# Autodesk Inventor assembly: ImpresionGrua
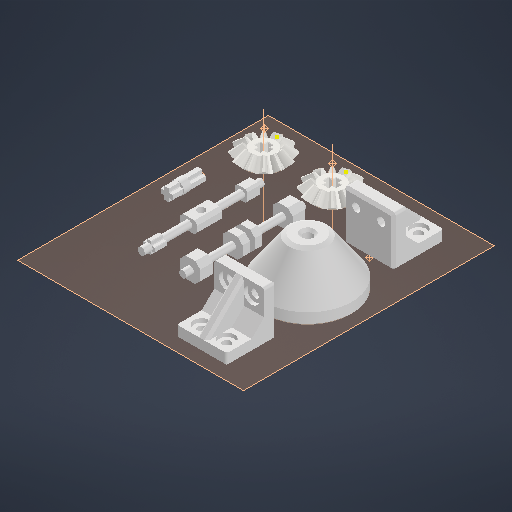
[picture p0: Inventor's stored thumbnail of the model, 512x512]
Saved by Autodesk Inventor 2026.3 (Build 303398000, 398)
## iProperties
Created: 2026-05-15
Part Number: ImpresionGrua
Document SubType Name: Assembly
Designer: Caro
Author: Caro
## Documents named in this file (7)
- C:\Users\Caro\JoseCarlos\TEC\TFG\Inventor\PiezasSTD\EnsamblesDeImpresion\ImpresionGrua.iam
- C:\Users\Caro\JoseCarlos\TEC\TFG\Inventor\PiezasSTD\EnsambleGarraSTD\Design Accelerator\Engranaje biselado11.ipt
- C:\Users\Caro\JoseCarlos\TEC\TFG\Inventor\PiezasSTD\EnsambleGruaSTD\EjeCortoGrua.ipt
- C:\Users\Caro\JoseCarlos\TEC\TFG\Inventor\PiezasSTD\EnsambleGruaSTD\EjeEngraneGrua.ipt
- C:\Users\Caro\JoseCarlos\TEC\TFG\Inventor\PiezasSTD\EnsambleGruaSTD\EjeFrontalGrúa.ipt
- C:\Users\Caro\JoseCarlos\TEC\TFG\Inventor\PiezasSTD\EnsambleGruaSTD\PesaGrua.ipt
- C:\Users\Caro\JoseCarlos\TEC\TFG\Inventor\PiezasSTD\T.ipt
## Components (8 placed, 6 different names)
1. Engranaje biselado1:1 — Coincidencia:1
2. Engranaje biselado1:2 — Coincidencia:2
3. EjeCortoGrua:1 — Coincidencia:3
4. EjeEngraneGrua:1 — Coincidencia:4
5. EjeFrontalGrúa:1 — Coincidencia:5
6. PesaGrua:1 — Coincidencia:8
7. T:1 — Coincidencia:6, Ángulo:1
8. T:2 — Coincidencia:7, Ángulo:1
## Relationships (9: Mate 8, Angle 1)
- Coincidencia:1 [Mate]: Engranaje biselado1:1
- Coincidencia:2 [Mate]: Engranaje biselado1:2
- Coincidencia:3 [Mate]: EjeCortoGrua:1
- Coincidencia:4 [Mate]: EjeEngraneGrua:1
- Coincidencia:5 [Mate]: EjeFrontalGrúa:1
- Coincidencia:6 [Mate]: T:1
- Coincidencia:7 [Mate]: T:2
- Ángulo:1 [Angle] (180 deg): T:1 ↔ T:2
- Coincidencia:8 [Mate]: PesaGrua:1
